# Autodesk Inventor assembly: AA00001149390 Assy Corrugated
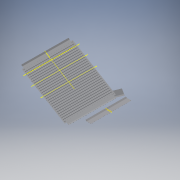
[picture p0: Inventor's stored thumbnail of the model, 180x180]
Saved by Autodesk Inventor 2017 (Build 210142000, 142)
## iProperties
Created: 2019-04-12
Part Number: AA00001149390 Assy Corrugated
Document SubType Name: Assembly
Designer: Phs
Author: Phs
## Documents named in this file (8)
- C:\Users\Phs\Documents\Inventor\Eriyeti Murena\Assy Corrugated\AA00001149390 Assy Corrugated.iam
- C:\Users\Phs\Documents\Inventor\Eriyeti Murena\Assy Corrugated\AAD0001104381.ipt
- C:\Users\Phs\Documents\Inventor\Eriyeti Murena\Assy Corrugated\AAD0001101755.ipt
- C:\Users\Phs\Documents\Inventor\Eriyeti Murena\Assy Corrugated\AAD0001038936.ipt
- C:\Users\Phs\Documents\Inventor\Eriyeti Murena\Assy Corrugated\AAD0001038947.ipt
- C:\Users\Phs\Documents\Inventor\Eriyeti Murena\Assy Corrugated\AAD0001104381_MIR.ipt
- C:\Users\Phs\Documents\Inventor\Eriyeti Murena\Assy Corrugated\AAD0001101755_MIR.ipt
- C:\Users\Phs\Documents\Inventor\Eriyeti Murena\Assy Corrugated\AAD0001038936_MIR.ipt
## Components (9 placed, 7 different names)
1. AAD0001104381:1
2. AAD0001104381:2 — Mate:1, Flush:1, Mate:2
3. AAD0001101755:1 — Mate:1, Flush:1, Mate:2, Mate:3, Flush:2, Mate:4
4. AAD0001038936:1 — Mate:3, Flush:2, Mate:4, Mate:5, Flush:3, Mate:6
5. AAD0001038947:1 — Mate:5, Flush:3, Mate:6
6. AAD0001104381_MIR:1
7. AAD0001104381_MIR:2 — Mate:7, Flush:4, Mate:8
8. AAD0001101755_MIR:1 — Mate:7, Flush:4, Mate:8, Mate:9, Flush:5, Mate:10
9. AAD0001038936_MIR:1 — Mate:9, Flush:5, Mate:10
## Relationships (15: Mate 10, Flush 5)
- Mate:1: AAD0001104381:2 ↔ AAD0001101755:1
- Flush:1: AAD0001104381:2 ↔ AAD0001101755:1
- Mate:2 (-106.865 mm): AAD0001104381:2 ↔ AAD0001101755:1
- Mate:3: AAD0001101755:1 ↔ AAD0001038936:1
- Flush:2: AAD0001101755:1 ↔ AAD0001038936:1
- Mate:4 (-30 mm): AAD0001101755:1 ↔ AAD0001038936:1
- Mate:5: AAD0001038936:1 ↔ AAD0001038947:1
- Flush:3: AAD0001038936:1 ↔ AAD0001038947:1
- Mate:6 (-30 mm): AAD0001038936:1 ↔ AAD0001038947:1
- Mate:7 (-106.865 mm): AAD0001104381_MIR:2 ↔ AAD0001101755_MIR:1
- Flush:4: AAD0001104381_MIR:2 ↔ AAD0001101755_MIR:1
- Mate:8: AAD0001104381_MIR:2 ↔ AAD0001101755_MIR:1
- Mate:9 (-30 mm): AAD0001101755_MIR:1 ↔ AAD0001038936_MIR:1
- Flush:5: AAD0001101755_MIR:1 ↔ AAD0001038936_MIR:1
- Mate:10: AAD0001101755_MIR:1 ↔ AAD0001038936_MIR:1
